# Autodesk Inventor assembly: Ball Shifter 110mm Shaft assy
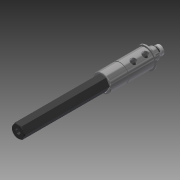
[picture p0: Inventor's stored thumbnail of the model, 180x180]
Saved by Autodesk Inventor 2013 (Build 170138000, 138)
## iProperties
Created: 2013-04-08
Part Number: Ball Shifter 110mm Shaft assy
Document SubType Name: Assembly
Designer: Niemitalo_Dan
Author: Niemitalo_Dan
## Documents named in this file (6)
- \\lmss\students\Robotics\CAD Files\COTS Parts\Gearboxes\Components\VexPro Ball Shifters\Ball Shifter 110mm Shaft assy.iam
- \\lmss\students\Robotics\CAD Files\COTS Parts\Gearboxes\Components\VexPro Ball Shifters\BallShifter ball housing.ipt
- \\lmss\students\Robotics\CAD Files\COTS Parts\Gearboxes\Components\VexPro Ball Shifters\Ball shifting shaft.ipt
- \\lmss\students\Robotics\CAD Files\COTS Parts\Gearboxes\Components\VexPro Ball Shifters\Shifter shaft bearing.ipt
- \\lmss\students\Robotics\CAD Files\COTS Parts\Gearboxes\Components\VexPro Ball Shifters\Shifter shaft small clip ring.ipt
- \\lmss\students\Robotics\CAD Files\COTS Parts\Gearboxes\Components\VexPro Ball Shifters\Ballshifter Long 110mm Output Shaft.ipt
## Components (6 placed, 5 different names)
1. BallShifter ball housing:1 — Mate:1, Mate:2, Angle:1, Mate:3, Flush:1
2. Ball shifting shaft:1 — Mate:1, Flush:1, Insert:1, Insert:2, Insert:3
3. Ballshifter Long 110mm Output Shaft:1 — Mate:2, Angle:1, Mate:3
4. Shifter shaft ring:1 — Insert:3
5. Shifter shaft small clip ring:1 — Insert:2
6. Shifter shaft small clip ring:2 — Insert:1
## Relationships (8: Mate 3, Insert 3, Angle 1, Flush 1)
- Mate:1: BallShifter ball housing:1 ↔ Ball shifting shaft:1
- Mate:2: BallShifter ball housing:1 ↔ Ballshifter Long 110mm Output Shaft:1
- Angle:1 (0 deg): BallShifter ball housing:1 ↔ Ballshifter Long 110mm Output Shaft:1
- Mate:3: BallShifter ball housing:1 ↔ Ballshifter Long 110mm Output Shaft:1
- Flush:1 (8.382 mm): BallShifter ball housing:1 ↔ Ball shifting shaft:1
- Insert:1: Ball shifting shaft:1 ↔ Shifter shaft small clip ring:2
- Insert:2: Ball shifting shaft:1 ↔ Shifter shaft small clip ring:1
- Insert:3: Ball shifting shaft:1 ↔ Shifter shaft ring:1
